# Autodesk Inventor assembly: Test Section
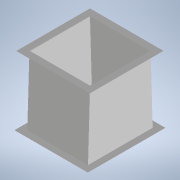
[picture p0: Inventor's stored thumbnail of the model, 180x180]
Saved by Autodesk Inventor 2022 (Build 260153000, 153)
## iProperties
Created: 2022-03-07
Part Number: Test Section
Document SubType Name: Assembly
Designer: calvi
Author: calvi
## Documents named in this file (4)
- E:\Dr. A Muchiri\Wind tunnel_Dr.A Muchiri\Test Section.iam
- E:\Dr. A Muchiri\Wind tunnel_Dr.A Muchiri\Test Section Frame.ipt
- E:\Dr. A Muchiri\Wind tunnel_Dr.A Muchiri\Test Section Ver2 Frame.ipt
- E:\Dr. A Muchiri\Wind tunnel_Dr.A Muchiri\Test Section Ver2.ipt
## Components (3 placed, 3 different names)
1. Test Section Frame:1 — Mate:1, Mate:2
2. Test Section Ver2 Frame:1 — Mate:3, Mate:4
3. Test Section Ver2:1 — Mate:1, Mate:2, Mate:3, Mate:4
## Relationships (4: Mate 4)
- Mate:1: Test Section Frame:1 ↔ Test Section Ver2:1
- Mate:2: Test Section Frame:1 ↔ Test Section Ver2:1
- Mate:3: Test Section Ver2 Frame:1 ↔ Test Section Ver2:1
- Mate:4: Test Section Ver2 Frame:1 ↔ Test Section Ver2:1
